# Autodesk Inventor assembly: Ventilador
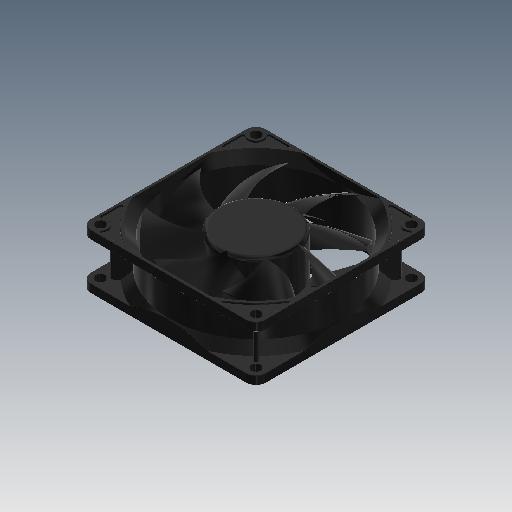
[picture p0: Inventor's stored thumbnail of the model, 512x512]
Saved by Autodesk Inventor 2020 (Build 240168000, 168)
## iProperties
Created: 2020-06-28
Part Number: Ventilador
Document SubType Name: Assembly
Designer: Dante
Author: Dante
## Documents named in this file (3)
- C:\Users\Usuario\Desktop\Ensamble Ajust Fino Total + Elect. - Act. 19_10_2020 - copia\Componentes Electrónicos\Cooler 80x80x25\pc-fan-19.snapshot.1\Ventilador.iam
- C:\Users\Usuario\Desktop\Ensamble Ajust Fino Total + Elect. - Act. 19_10_2020 - copia\Componentes Electrónicos\Cooler 80x80x25\pc-fan-19.snapshot.1\PC fan.ipt
- C:\Users\Usuario\Desktop\Ensamble Ajust Fino Total + Elect. - Act. 19_10_2020 - copia\Componentes Electrónicos\Cooler 80x80x25\pc-fan-19.snapshot.1\PC fan_part 2.ipt
## Components (2 placed, 2 different names)
1. PC fan:1 — Mate:1, Mate:2
2. PC fan_part 2:1 — Mate:1, Mate:2
## Relationships (2: Mate 2)
- Mate:1: PC fan:1 ↔ PC fan_part 2:1
- Mate:2 (3.5 mm): PC fan:1 ↔ PC fan_part 2:1
